# Autodesk Inventor assembly: interiorElectronics
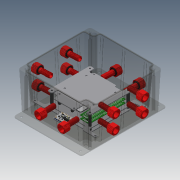
[picture p0: Inventor's stored thumbnail of the model, 180x180]
Saved by Autodesk Inventor 2018 (Build 220112000, 112)
## iProperties
Created: 2020-02-05
Part Number: interiorElectronics
Document SubType Name: Assembly
Designer: anirudh
Author: anirudh
## Documents named in this file (3)
- D:\Silicon Sharks\2019-2020\ElectronicsHousing\Prototype3\interiorElectronics.iam
- D:\Silicon Sharks\2019-2020\ElectronicsHousing\Prototype3\mainEnclosure.iam
- D:\Silicon Sharks\2019-2020\ElectronicsHousing\Prototype3\electronicsLayout.iam
## Components (2 placed, 2 different names)
1. mainEnclosure:1 [sub-assembly] — Mate:1, Mate:2
2. electronicsLayout:1 [sub-assembly] — Mate:1, Mate:2
## Relationships (2: Mate 2)
- Mate:1: mainEnclosure:1 ↔ electronicsLayout:1
- Mate:2: mainEnclosure:1 ↔ electronicsLayout:1
